# Autodesk Inventor assembly: motor_frontalholder_combo
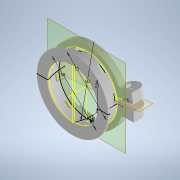
[picture p0: Inventor's stored thumbnail of the model, 180x180]
Saved by Autodesk Inventor 2020 (Build 240168000, 168)
## iProperties
Created: 2019-08-02
Part Number: motor_frontalholder_combo
Document SubType Name: Assembly
Designer: erwin
Author: erwin
## Documents named in this file (3)
- D:\GitHub\BeachMaid\platform\motor_frontalholder_combo.iam
- D:\GitHub\BeachMaid\platform\motor_frontalholder.ipt
- D:\GitHub\BeachMaid\platform\motor_frontalholder_retainerscrew.ipt
## Components (2 placed, 2 different names)
1. motor_frontalholder:1 — Flush:1
2. motor_frontalholder_retainerscrew:1 — Flush:1
## Relationships (1: Flush 1)
- Flush:1: motor_frontalholder:1 ↔ motor_frontalholder_retainerscrew:1
